# Autodesk Inventor assembly: Placed 180 deg corner cabinet
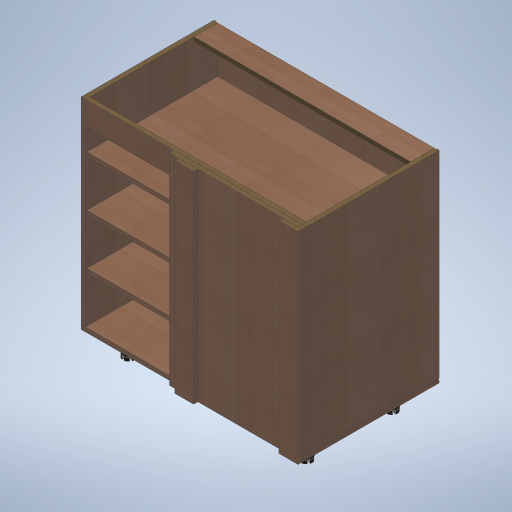
[picture p0: Inventor's stored thumbnail of the model, 512x512]
Saved by Autodesk Inventor 2024 (Build 280153000, 153)
## iProperties
RuleStatus: InUse
Created: 2017-02-02
Part Number: Placed 180 deg corner cabinet
Document SubType Name: Assembly
Designer: SvetlanaB
Author: SvetlanaB
## Documents named in this file (22)
- C:\W4INV 2024 Design\iBOX LIBRARY\Kitchen\Standing Cabinets\180 deg corner cabinet\180 deg Corner Cabinet.iam
- C:\W4INV 2024 Design\iBOX LIBRARY\Kitchen\Standing Cabinets\180 deg corner cabinet\Right panel.ipt
- C:\W4INV 2024 Design\iBOX LIBRARY\Kitchen\Standing Cabinets\180 deg corner cabinet\Left panel.ipt
- C:\W4INV 2024 Design\iBOX LIBRARY\Kitchen\Standing Cabinets\180 deg corner cabinet\Bottom panel.ipt
- C:\W4INV 2024 Design\iBOX LIBRARY\Kitchen\Standing Cabinets\180 deg corner cabinet\Skeleton Panel1.ipt
- C:\W4INV 2024 Design\iBOX LIBRARY\Kitchen\Standing Cabinets\180 deg corner cabinet\Back panel.ipt
- C:\W4INV 2024 Design\iBOX LIBRARY\Kitchen\Standing Cabinets\180 deg corner cabinet\Back top panel.ipt
- C:\W4INV 2024 Design\iBOX LIBRARY\Kitchen\Standing Cabinets\180 deg corner cabinet\Front top panel.ipt
- C:\W4INV 2024 Design\iBOX LIBRARY\Kitchen\Standing Cabinets\180 deg corner cabinet\Front panel.ipt
- C:\W4INV 2024 Design\iBOX LIBRARY\Kitchen\Standing Cabinets\180 deg corner cabinet\Front small panel.ipt
- C:\W4INV 2024 Design\_LIBRARY\Supports and legs\Legs\ADJUSTABLE LEG\Adjustable leg  BT18 clip included.ipt
- C:\W4INV 2024 Design\_LIBRARY\Holders\Shelf holder D5\Shelf support D5 L16 with hole covers.ipt
- C:\W4INV 2024 Design\_LIBRARY\Supports and legs\Legs\ADJUSTABLE LEG\Adjustable leg  BT18.ipt
- C:\W4INV 2024 Design\_LIBRARY\Fixed joints\Confirmat\CONFIRMAT\Confirmat L50 NB T18 PB T 18.ipt
- C:\W4INV 2024 Design\iBOX LIBRARY\Kitchen\Standing Cabinets\180 deg corner cabinet\corner cabinet concept.ipt
- C:\W4INV 2024 Design\_LIBRARY\Fixed joints\Minifix joint\MINIFIX D15 v2\Minifix D15 & Dowel L34 & Cap D15 PB T18 LH.ipt
- C:\W4INV 2024 Design\_LIBRARY\Fixed joints\Minifix joint\MINIFIX D15 v2\Minifix D15 & Dowel L34 & Cap D15 PB T18 RH.ipt
- C:\W4INV 2024 Design\_LIBRARY\Fixed joints\Confirmat\CONFIRMAT\Confirmat L50 & Cap D10 NB T18 PB T 18.ipt
- C:\W4INV 2023 Design\LIBRARY\Fixed joints\Confirmat\CONFIRMAT.ipt
- C:\W4INV 2023 Design\LIBRARY\Fixed joints\Minifix joint\MINIFIX D15 v2.ipt
- C:\W4INV 2023 Design\LIBRARY\Holders\Shelf holder D5.ipt
- C:\W4INV 2023 Design\LIBRARY\Supports and legs\Legs\ADJUSTABLE LEG.ipt
## Components (38 placed, 17 different names)
1. @Skeleton
2. Right panel:1 — Side Board Plane:1, Side Board Plane:2, Pillar Board Side Plane:2, Pillar Board Side Plane:4, Nestled Board Plane:8, Nestled Board Plane:5, Mate:99, Flush:43, Flush:44, Mate:100
3. Left panel:1 — Flush:5, Flush:6, Side Board Plane:3, Side Board Plane:4, Nestled Board Plane:10, Nestled Board Plane:9, Nestled Board Plane:6, Pillar Board Side Plane:1, Pillar Board Side Plane:3, Mate:101, Flush:45
4. Bottom panel:1 — Flush:1, Flush:2, Flush:3, Flush:4, Bottom board Plane:1, Front (Angle) Plane:1, Bottom board Plane:2, Front (Angle) Plane:2, Bottom board Plane:3, Front (Angle) Plane:3, Bottom board Plane:4, Front (Angle) Plane:4, Nestled Board Plane:2, Nestled Board Plane:4, Nestled Board Plane:1, Nestled Board Plane:3
5. Back panel:1 — Mate:100, Mate:101, Flush:45
6. Back top panel:1 — Flush:27, Pillar Board Side Plane:10, Pillar Board Side Plane :5, Pillar Board Side Plane :6, Mate:99, Flush:43, Flush:44
7. Front top panel:1 — Flush:11, Pillar Board Side Plane :7, Pillar Board Side Plane :8
8. Front panel:1 — Flush:17, Flush:18, Mate:53
9. Front small panel:1
10. Adjustable leg  BT18 clip included:1 — Axis2 Plane:1, Axis Plane:1, Bottom board Plane:1, Front (Angle) Plane:1
11. Adjustable leg  BT18 clip included:2 — Axis2 Plane:2, Axis Plane:2, Bottom board Plane:2, Front (Angle) Plane:2
12. Adjustable leg  BT18:3 — Axis2 Plane:3, Axis Plane:3, Bottom board Plane:3, Front (Angle) Plane:3
13. Adjustable leg  BT18:4 — Axis2 Plane:4, Axis Plane:4, Bottom board Plane:4, Front (Angle) Plane:4
14. Front small panel:2 — Flush:17, Flush:18, Mate:53
15. Confirmat L50 & Cap D10 NB T18 PB T 18:2 — Axis Plane:6, Pillar Board Side Plane:2, Nestled Board Plane:2
16. Confirmat L50 NB T18 PB T 18:4 — Axis Plane:8, Pillar Board Side Plane:4, Nestled Board Plane:4
17. Confirmat L50 NB T18 PB T 18:10 — Nestled Board Plane:10, Pillar Board Side Plane:10, Axis Plane:18
18. Minifix D15 & Dowel L34 & Cap D15 PB T18 RH:5 — Nestled Board Plane:8, Pillar Board Side Plane :5, Axis Plane:15
19. Minifix D15 & Dowel L34 & Cap D15 PB T18 LH:6 — Nestled Board Plane:9, Pillar Board Side Plane :6, Axis Plane:16
20. Minifix D15 & Dowel L34 & Cap D15 PB T18 RH:7 — Nestled Board Plane:5, Pillar Board Side Plane :7, Axis Plane:13
21. Minifix D15 & Dowel L34 & Cap D15 PB T18 LH:8 — Nestled Board Plane:6, Pillar Board Side Plane :8, Axis Plane:14
22. Confirmat L50 NB T18 PB T 18:11 — Axis Plane:5, Nestled Board Plane:1, Pillar Board Side Plane:1
23. Confirmat L50 NB T18 PB T 18:12 — Axis Plane:7, Nestled Board Plane:3, Pillar Board Side Plane:3
24. Skeleton Panel1:1 — Shelf Pottom Plane:1, Shelf Pottom Plane:2, Shelf Pottom Plane:3, Shelf Pottom Plane:4
25. Shelf support D5 L16 with hole covers:3 — Axis Plane:11, Side Board Plane:3, Shelf Pottom Plane:3
26. Shelf support D5 L16 with hole covers:4 — Axis Plane:12, Side Board Plane:4, Shelf Pottom Plane:4
27. Shelf support D5 L16 with hole covers:2 — Axis Plane:10, Side Board Plane:2, Shelf Pottom Plane:2
28. Shelf support D5 L16 with hole covers:1 — Axis Plane:9, Side Board Plane:1, Shelf Pottom Plane:1
29. Skeleton Panel1:2
30. Shelf support D5 L16 with hole covers:5
31. Shelf support D5 L16 with hole covers:6
32. Shelf support D5 L16 with hole covers:7
33. Shelf support D5 L16 with hole covers:8
34. Skeleton Panel1:3
35. Shelf support D5 L16 with hole covers:9
36. Shelf support D5 L16 with hole covers:10
37. Shelf support D5 L16 with hole covers:11
38. Shelf support D5 L16 with hole covers:12
## Component patterns: (3 elements, first: Skeleton Panel1:1 + Shelf support D5 L16 with hole covers:3 + Shelf support D5 L16 with hole covers:4 + Shelf support D5 L16 with hole covers:2 + Shelf support D5 L16 with hole covers:1)
## Relationships (72: Mate 46, Flush 22, Angle 4)
- Flush:1 (-100 mm): Bottom panel:1
- Flush:2 (-100 mm): Bottom panel:1
- Flush:3 (-100 mm): Bottom panel:1
- Flush:4 (-100 mm): Bottom panel:1
- Flush:5 (-64 mm): Left panel:1
- Flush:6 (-64 mm): Left panel:1
- Axis Plane:9 [Mate]: Shelf support D5 L16 with hole covers:1
- Side Board Plane:1 [Mate]: Right panel:1 ↔ Shelf support D5 L16 with hole covers:1
- Shelf Pottom Plane:1 [Mate] (2.5 mm): Skeleton Panel1:1 ↔ Shelf support D5 L16 with hole covers:1
- Axis Plane:10 [Mate]: Shelf support D5 L16 with hole covers:2
- Side Board Plane:2 [Mate]: Right panel:1 ↔ Shelf support D5 L16 with hole covers:2
- Shelf Pottom Plane:2 [Mate] (2.5 mm): Skeleton Panel1:1 ↔ Shelf support D5 L16 with hole covers:2
- Axis Plane:11 [Mate]: Shelf support D5 L16 with hole covers:3
- Side Board Plane:3 [Mate]: Left panel:1 ↔ Shelf support D5 L16 with hole covers:3
- Shelf Pottom Plane:3 [Mate] (2.5 mm): Skeleton Panel1:1 ↔ Shelf support D5 L16 with hole covers:3
- Axis Plane:12 [Mate]: Shelf support D5 L16 with hole covers:4
- Side Board Plane:4 [Mate]: Left panel:1 ↔ Shelf support D5 L16 with hole covers:4
- Shelf Pottom Plane:4 [Mate] (2.5 mm): Skeleton Panel1:1 ↔ Shelf support D5 L16 with hole covers:4
- Flush:11 (-50 mm): Front top panel:1
- Axis2 Plane:1 [Mate]: Adjustable leg  BT18 clip included:1
- Axis Plane:1 [Mate]: Adjustable leg  BT18 clip included:1
- Bottom board Plane:1 [Mate]: Bottom panel:1 ↔ Adjustable leg  BT18 clip included:1
- Front (Angle) Plane:1 [Angle] (0 deg): Bottom panel:1 ↔ Adjustable leg  BT18 clip included:1
- Axis2 Plane:2 [Mate]: Adjustable leg  BT18 clip included:2
- Axis Plane:2 [Mate]: Adjustable leg  BT18 clip included:2
- Bottom board Plane:2 [Mate]: Bottom panel:1 ↔ Adjustable leg  BT18 clip included:2
- Front (Angle) Plane:2 [Angle] (0 deg): Bottom panel:1 ↔ Adjustable leg  BT18 clip included:2
- Axis2 Plane:3 [Mate]: Adjustable leg  BT18:3
- Axis Plane:3 [Mate]: Adjustable leg  BT18:3
- Bottom board Plane:3 [Mate]: Bottom panel:1 ↔ Adjustable leg  BT18:3
- Front (Angle) Plane:3 [Angle] (0 deg): Bottom panel:1 ↔ Adjustable leg  BT18:3
- Axis2 Plane:4 [Mate]: Adjustable leg  BT18:4
- Axis Plane:4 [Mate]: Adjustable leg  BT18:4
- Bottom board Plane:4 [Mate]: Bottom panel:1 ↔ Adjustable leg  BT18:4
- Front (Angle) Plane:4 [Angle] (0 deg): Bottom panel:1 ↔ Adjustable leg  BT18:4
- Flush:17: Front panel:1 ↔ Front small panel:2
- Flush:18: Front panel:1 ↔ Front small panel:2
- Mate:53: Front panel:1 ↔ Front small panel:2
- Axis Plane:6 [Mate]: Confirmat L50 & Cap D10 NB T18 PB T 18:2
- Pillar Board Side Plane:2 [Mate] (-9 mm): Right panel:1 ↔ Confirmat L50 & Cap D10 NB T18 PB T 18:2
- Nestled Board Plane:2 [Flush]: Bottom panel:1 ↔ Confirmat L50 & Cap D10 NB T18 PB T 18:2
- Axis Plane:8 [Mate]: Confirmat L50 NB T18 PB T 18:4
- Pillar Board Side Plane:4 [Mate] (-9 mm): Right panel:1 ↔ Confirmat L50 NB T18 PB T 18:4
- Nestled Board Plane:4 [Flush]: Bottom panel:1 ↔ Confirmat L50 NB T18 PB T 18:4
- Flush:27 (-70 mm): Back top panel:1
- Nestled Board Plane:10 [Flush]: Left panel:1 ↔ Confirmat L50 NB T18 PB T 18:10
- Pillar Board Side Plane:10 [Mate] (-9 mm): Back top panel:1 ↔ Confirmat L50 NB T18 PB T 18:10
- Axis Plane:18 [Mate]: Confirmat L50 NB T18 PB T 18:10
- Nestled Board Plane:8 [Mate]: Right panel:1 ↔ Minifix D15 & Dowel L34 & Cap D15 PB T18 RH:5
- Pillar Board Side Plane :5 [Flush] (18 mm): Back top panel:1 ↔ Minifix D15 & Dowel L34 & Cap D15 PB T18 RH:5
- Axis Plane:15 [Mate]: Minifix D15 & Dowel L34 & Cap D15 PB T18 RH:5
- Nestled Board Plane:9 [Mate]: Left panel:1 ↔ Minifix D15 & Dowel L34 & Cap D15 PB T18 LH:6
- Pillar Board Side Plane :6 [Flush] (18 mm): Back top panel:1 ↔ Minifix D15 & Dowel L34 & Cap D15 PB T18 LH:6
- Axis Plane:16 [Mate]: Minifix D15 & Dowel L34 & Cap D15 PB T18 LH:6
- Nestled Board Plane:5 [Mate]: Right panel:1 ↔ Minifix D15 & Dowel L34 & Cap D15 PB T18 RH:7
- Pillar Board Side Plane :7 [Flush] (18 mm): Front top panel:1 ↔ Minifix D15 & Dowel L34 & Cap D15 PB T18 RH:7
- Axis Plane:13 [Mate]: Minifix D15 & Dowel L34 & Cap D15 PB T18 RH:7
- Nestled Board Plane:6 [Mate]: Left panel:1 ↔ Minifix D15 & Dowel L34 & Cap D15 PB T18 LH:8
- Pillar Board Side Plane :8 [Flush] (18 mm): Front top panel:1 ↔ Minifix D15 & Dowel L34 & Cap D15 PB T18 LH:8
- Axis Plane:14 [Mate]: Minifix D15 & Dowel L34 & Cap D15 PB T18 LH:8
- Axis Plane:5 [Mate]: Confirmat L50 NB T18 PB T 18:11
- Nestled Board Plane:1 [Flush]: Bottom panel:1 ↔ Confirmat L50 NB T18 PB T 18:11
- Pillar Board Side Plane:1 [Mate] (-9 mm): Left panel:1 ↔ Confirmat L50 NB T18 PB T 18:11
- Axis Plane:7 [Mate]: Confirmat L50 NB T18 PB T 18:12
- Nestled Board Plane:3 [Flush]: Bottom panel:1 ↔ Confirmat L50 NB T18 PB T 18:12
- Pillar Board Side Plane:3 [Mate] (-9 mm): Left panel:1 ↔ Confirmat L50 NB T18 PB T 18:12
- Mate:99: Right panel:1 ↔ Back top panel:1
- Flush:43: Right panel:1 ↔ Back top panel:1
- Flush:44: Right panel:1 ↔ Back top panel:1
- Mate:100: Right panel:1 ↔ Back panel:1
- Mate:101 (0.5 mm): Left panel:1 ↔ Back panel:1
- Flush:45: Left panel:1 ↔ Back panel:1
## Named parameters: Panel_thickness = 18 mm, Shelf_quantity = 3, Front_panel_position = 560 mm, Shelf_position = 194.5 mm
